# Autodesk Inventor assembly: Робот RRO 2021
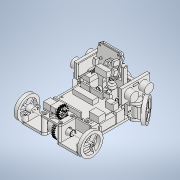
[picture p0: Inventor's stored thumbnail of the model, 180x180]
Saved by Autodesk Inventor 2020 (Build 240168000, 168)
## iProperties
Created: 2021-02-28
Part Number: Робот RRO 2021
Document SubType Name: Assembly
Designer: Антон
Author: Антон
## Documents named in this file (44)
- D:\Project\Robots\RRO 2021\Робот RRO 2021.iam
- D:\Project\Robots\RRO 2021\Body\Основа робота.ipt
- D:\Project\Robots\RRO 2021\Components\Кронштейн для двигателей серии N.ipt
- D:\Project\Robots\RRO 2021\Components\Servo SG90.ipt
- D:\Project\Robots\RRO 2021\Body\Основа рулевого механизма.ipt
- D:\Project\Robots\RRO 2021\Components\Подшипники\Подшипник 3 8 3.ipt
- D:\Project\Robots\RRO 2021\Components\Оси\Ось 3мм рулевого управления.ipt
- D:\Project\Robots\RRO 2021\Body\Деталь крепления диска к поворотному механизму.ipt
- D:\Project\Robots\RRO 2021\Components\Оси\Ось 3мм колеса.ipt
- D:\Project\Robots\RRO 2021\Body\Втулка между подшипниками рулевого управления.ipt
- D:\Project\Robots\RRO 2021\Components\Оси\Ось балки рулевого управления ведущая.ipt
- D:\Project\Robots\RRO 2021\Body\Балка рулевого управления ведущая.ipt
- D:\Project\Robots\RRO 2021\Body\Деталь крепления диска к поворотному механизму_ЗЕРКАЛО1.ipt
- D:\Project\Robots\RRO 2021\Body\Стойка под электроннику.ipt
- D:\Project\Robots\RRO 2021\Components\Arduino UNO.ipt
- D:\Project\Robots\RRO 2021\Body\Крепление камеры.ipt
- D:\Project\Robots\RRO 2021\Components\nVision lipo battery.ipt
- D:\Project\Robots\RRO 2021\Components\Micro Gearmotors.ipt
- D:\Project\Robots\RRO 2021\Components\Trackingcam (Applied robotics).ipt
- D:\Project\Robots\RRO 2021\Body\Стойка для камеры.ipt
- D:\Project\Robots\RRO 2021\Components\Подшипники\Подшипник 2 5 2,5.ipt
- D:\Project\Robots\RRO 2021\Components\Оси\Ось 2мм рулевой сервы.ipt
- D:\Project\Robots\RRO 2021\Body\Поворотный рычаг для сервы.ipt
- D:\Project\Robots\RRO 2021\Body\Крышка стойки подшипника 3мм.ipt
- D:\Project\Robots\RRO 2021\Body\Стойки камеры.ipt
- D:\Project\Robots\RRO 2021\Body\Съемная стойка сервы.ipt
- D:\Project\Robots\RRO 2021\Body\Крышка поворотного кулака.ipt
- D:\Project\Robots\RRO 2021\Components\Ultrasonic HC-SRO4.ipt
- D:\Project\Robots\RRO 2021\Body\Крышка аккумулятора.ipt
- D:\Project\Robots\RRO 2021\Body\Стойка подшипника 3мм.ipt
- D:\Project\Robots\RRO 2021\Components\Оси\Ось 3мм задняя.ipt
- D:\Project\Robots\RRO 2021\Body\Крепление ультрасоника.ipt
- D:\Project\Robots\RRO 2021\Body\Крепление ультрасоника вертикальная.ipt
- D:\Project\Robots\RRO 2021\Body\Крепление ультрасоника вертикальная_ЗЕРКАЛО.ipt
- D:\Project\Robots\RRO 2021\Components\Дифференциал.ipt
- D:\Project\Robots\RRO 2021\Body\Ведущая шестерня дифференециала.ipt
- D:\Project\Robots\RRO 2021\Components\Подшипники\Подшипник 10 15 4.ipt
- D:\Project\Robots\RRO 2021\Body\Переходник с дифференциала на ось 3мм.ipt
- D:\Project\Robots\RRO 2021\Components\Оси\Ось мотора серии N.ipt
- D:\Project\Robots\RRO 2021\Body\Крепление дифференциала.ipt
- D:\Project\Robots\RRO 2021\Body\Крепление двигателя2.ipt
- D:\Project\Robots\RRO 2021\Body\Проставка для двигателя.ipt
- D:\Project\Robots\RRO 2021\Components\Колесо D40 под ось моторов серии N.ipt
- D:\Project\Robots\RRO 2021\Body\Деталь основы рулевого управления.ipt
## Components (75 placed, 43 different names)
1. Основа робота:1 — Жесткий:138, Жесткий:152, Жесткий:153, Жесткий:189, Жесткий:190, Жесткий:195, Жесткий:203
2. Основа рулевого механизма:1 — Жесткий:45, С поворотом:161, Жесткий:181, Жесткий:186, Жесткий:195, Жесткий:201, Жесткий:202, Жесткий:204, Жесткий:208, Жесткий:209
3. Съемная стойка сервы:1 — Жесткий:186
4. Servo SG90:2 — Жесткий:181, С поворотом:163
5. Поворотный рычаг для сервы:1 — С поворотом:163, Жесткий:183
6. Подшипник 2*5*2.5:2 — С поворотом:162, Жесткий:183
7. Ось 2мм рулевой сервы:1 — С поворотом:24, С поворотом:162
8. Подшипник 2*5*2.5:1 — С поворотом:24, Жесткий:184
9. Балка рулевого управления:1 — С поворотом:35, С поворотом:36, Жесткий:184
10. Деталь основы рулевого управления:2 — Жесткий:208
11. Деталь основы рулевого управления:1 — Жесткий:209
12. Крышка аккумулятора:1 — Жесткий:108
13. nVision lipo battery:1 — Жесткий:54
14. Стойка под электроннику:1 — Жесткий:53, Жесткий:54, Жесткий:108, Жесткий:203
15. Arduino UNO:1 — Жесткий:53
16. Ось 3мм задняя:2 — Жесткий:165, Жесткий:197
17. Крепление двигателя2:1 — Жесткий:191, Жесткий:194
18. Переходник с дифференциала на ось 3мм:1 — Жесткий:165, Жесткий:171
19. Дифференциал:1 — С поворотом:158, Жесткий:166, ЗубчПер:1, Жесткий:171, С поворотом:164
20. Переходник с дифференциала на ось 3мм:2 — Жесткий:166, Жесткий:170
21. Ось 3мм задняя:1 — Жесткий:170, Жесткий:196
22. Колесо D40 под ось моторов серии N:1 — Жесткий:196
23. Колесо D40 под ось моторов серии N:2 — Жесткий:199
24. Колесо D40 под ось моторов серии N:4 — Жесткий:197
25. Колесо D40 под ось моторов серии N:3 — Жесткий:198
26. Стойка для камеры:1 — С поворотом:32, Жесткий:204
27. Крышка поворотного кулака:2 — Жесткий:137
28. Деталь крепления диска к поворотному механизму:1 — Жесткий:13, Жесткий:14, Жесткий:34, Жесткий:125, Жесткий:137
29. Втулка между подшипниками рулевого управления:1 — Жесткий:11, Жесткий:12
30. Крышка поворотного кулака:1 — Жесткий:136
31. Деталь крепления диска к поворотному механизму_ЗЕРКАЛО1:1 — Жесткий:37, Жесткий:38, Жесткий:39, Жесткий:44, Жесткий:136
32. Втулка между подшипниками рулевого управления:2
33. Кронштейн для двигателей серии N:1 — Жесткий:174, Жесткий:193
34. Micro Gearmotors:1 — С поворотом:160, Жесткий:174
35. Проставка для двигателя:1 — Жесткий:193, Жесткий:194
36. Ось мотора серии N:1 — С поворотом:160, Жесткий:192
37. Ведущая шестерня дифференециала:1 — ЗубчПер:1, Жесткий:192
38. Крышка стойки подшипника 3мм:1 — Жесткий:109, Жесткий:110
39. Подшипник 3*8*3:9 — Жесткий:109
40. Стойка подшипника 3мм:1 — Жесткий:110, Жесткий:153
41. Крепление дифференциала:1 — Жесткий:188, Жесткий:189, Жесткий:191
42. Подшипник 10 15 4:1 — С поворотом:158, Жесткий:188
43. Крепление дифференциала:2 — Жесткий:190
44. Подшипник 10 15 4:2 — С поворотом:164
45. Крышка стойки подшипника 3мм:4 — Жесткий:114, Жесткий:163
46. Подшипник 3*8*3:10 — Жесткий:163
47. Стойка подшипника 3мм:4 — Жесткий:114, Жесткий:152
48. Крепление ультрасоника вертикальная_ЗЕРКАЛО:1 — Жесткий:202, Жесткий:205
49. Ultrasonic HC-SRO4:3 — Жесткий:205
50. Ultrasonic HC-SRO4:1 — Жесткий:207
51. Крепление ультрасоника горизонтальное:1 — Жесткий:138, Жесткий:207
52. Крепление ультрасоника вертикальное:1 — Жесткий:201, Жесткий:206
53. Ultrasonic HC-SRO4:2 — Жесткий:206
54. Trackingcam (Applied robotics):1 — Жесткий:95, Жесткий:96, Жесткий:97, Жесткий:98
55. Стойки камеры:1 — Жесткий:98
56. Стойки камеры:2 — Жесткий:95, Жесткий:99
57. Стойки камеры:3 — Жесткий:97
58. Стойки камеры:4 — Жесткий:96
59. Крепление камеры:1 — С поворотом:32, Жесткий:99
60. Ось 3мм рулевого управления:3 — С поворотом:14, Жесткий:14
61. Ось 3мм колеса:1 — С поворотом:12, Жесткий:199
62. Ось 3мм рулевого управления:1 — С поворотом:13, Жесткий:13
63. Ось балки рулевого управления ведущая:2 — Жесткий:34, С поворотом:35
64. Подшипник 3*8*3:1 — Жесткий:12
65. Подшипник 3*8*3:2 — С поворотом:13, Жесткий:45
66. Подшипник 3*8*3:3 — С поворотом:14
67. Подшипник 3*8*3:4 — Жесткий:11, С поворотом:12, Жесткий:125
68. Ось 3мм колеса:2 — Жесткий:198
69. Ось 3мм рулевого управления:4 — С поворотом:16, Жесткий:44
70. Ось балки рулевого управления ведущая:1 — Жесткий:39, С поворотом:36
71. Ось 3мм рулевого управления:5 — Жесткий:37
72. Подшипник 3*8*3:7
73. Подшипник 3*8*3:8 — Жесткий:38
74. Подшипник 3*8*3:6 — С поворотом:16, С поворотом:161
75. Подшипник 3*8*3:5
## Relationships (77: WeldJoint 60, RevoluteJoint 16, RelateRotation 1)
- Жесткий:11 [WeldJoint]: Втулка между подшипниками рулевого управления:1 ↔ Подшипник 3*8*3:4
- Жесткий:12 [WeldJoint]: Втулка между подшипниками рулевого управления:1 ↔ Подшипник 3*8*3:1
- С поворотом:12 [RevoluteJoint]: Ось 3мм колеса:1 ↔ Подшипник 3*8*3:4
- С поворотом:13 [RevoluteJoint]: Ось 3мм рулевого управления:1 ↔ Подшипник 3*8*3:2
- С поворотом:14 [RevoluteJoint]: Ось 3мм рулевого управления:3 ↔ Подшипник 3*8*3:3
- Жесткий:13 [WeldJoint]: Деталь крепления диска к поворотному механизму:1 ↔ Ось 3мм рулевого управления:1
- Жесткий:14 [WeldJoint]: Деталь крепления диска к поворотному механизму:1 ↔ Ось 3мм рулевого управления:3
- [WeldJoint]: Втулка между подшипниками рулевого управления:2 ↔ Подшипник 3*8*3:8
- [WeldJoint]: Втулка между подшипниками рулевого управления:2 ↔ Подшипник 3*8*3:5
- [RevoluteJoint]: Ось 3мм колеса:2 ↔ Подшипник 3*8*3:8
- С поворотом:16 [RevoluteJoint]: Ось 3мм рулевого управления:4 ↔ Подшипник 3*8*3:6
- [RevoluteJoint]: Ось 3мм рулевого управления:5 ↔ Подшипник 3*8*3:7
- Жесткий:34 [WeldJoint]: Деталь крепления диска к поворотному механизму:1 ↔ Ось балки рулевого управления ведущая:2
- Жесткий:37 [WeldJoint]: Деталь крепления диска к поворотному механизму_ЗЕРКАЛО1:1 ↔ Ось 3мм рулевого управления:5
- Жесткий:38 [WeldJoint]: Деталь крепления диска к поворотному механизму_ЗЕРКАЛО1:1 ↔ Подшипник 3*8*3:8
- Жесткий:39 [WeldJoint]: Деталь крепления диска к поворотному механизму_ЗЕРКАЛО1:1 ↔ Ось балки рулевого управления ведущая:1
- Жесткий:44 [WeldJoint]: Деталь крепления диска к поворотному механизму_ЗЕРКАЛО1:1 ↔ Ось 3мм рулевого управления:4
- Жесткий:45 [WeldJoint]: Основа рулевого механизма:1 ↔ Подшипник 3*8*3:2
- Жесткий:53 [WeldJoint]: Стойка под электроннику:1 ↔ Arduino UNO:1
- Жесткий:54 [WeldJoint]: nVision lipo battery:1 ↔ Стойка под электроннику:1
- С поворотом:24 [RevoluteJoint]: Ось 2мм рулевой сервы:1 ↔ Подшипник 2*5*2.5:1
- С поворотом:32 [RevoluteJoint] (-0.15 mm): Стойка для камеры:1 ↔ Крепление камеры:1
- Жесткий:95 [WeldJoint]: Trackingcam (Applied robotics):1 ↔ Стойки камеры:2
- Жесткий:96 [WeldJoint]: Trackingcam (Applied robotics):1 ↔ Стойки камеры:4
- Жесткий:97 [WeldJoint]: Trackingcam (Applied robotics):1 ↔ Стойки камеры:3
- Жесткий:98 [WeldJoint]: Trackingcam (Applied robotics):1 ↔ Стойки камеры:1
- Жесткий:99 [WeldJoint]: Стойки камеры:2 ↔ Крепление камеры:1
- Жесткий:108 [WeldJoint]: Крышка аккумулятора:1 ↔ Стойка под электроннику:1
- Жесткий:109 [WeldJoint] (-0.05 mm): Крышка стойки подшипника 3мм:1 ↔ Подшипник 3*8*3:9
- Жесткий:110 [WeldJoint]: Крышка стойки подшипника 3мм:1 ↔ Стойка подшипника 3мм:1
- Жесткий:114 [WeldJoint]: Крышка стойки подшипника 3мм:4 ↔ Стойка подшипника 3мм:4
- Жесткий:125 [WeldJoint]: Деталь крепления диска к поворотному механизму:1 ↔ Подшипник 3*8*3:4
- С поворотом:35 [RevoluteJoint]: Балка рулевого управления:1 ↔ Ось балки рулевого управления ведущая:2
- С поворотом:36 [RevoluteJoint]: Балка рулевого управления:1 ↔ Ось балки рулевого управления ведущая:1
- Жесткий:136 [WeldJoint]: Крышка поворотного кулака:1 ↔ Деталь крепления диска к поворотному механизму_ЗЕРКАЛО1:1
- Жесткий:137 [WeldJoint]: Крышка поворотного кулака:2 ↔ Деталь крепления диска к поворотному механизму:1
- Жесткий:138 [WeldJoint]: Основа робота:1 ↔ Крепление ультрасоника горизонтальное:1
- Жесткий:152 [WeldJoint]: Основа робота:1 ↔ Стойка подшипника 3мм:4
- Жесткий:153 [WeldJoint]: Основа робота:1 ↔ Стойка подшипника 3мм:1
- С поворотом:158 [RevoluteJoint] (-1 mm): Дифференциал:1 ↔ Подшипник 10 15 4:1
- Жесткий:163 [WeldJoint] (-0.05 mm): Крышка стойки подшипника 3мм:4 ↔ Подшипник 3*8*3:10
- Жесткий:165 [WeldJoint]: Ось 3мм задняя:2 ↔ Переходник с дифференциала на ось 3мм:1
- Жесткий:166 [WeldJoint]: Дифференциал:1 ↔ Переходник с дифференциала на ось 3мм:2
- Жесткий:170 [WeldJoint]: Переходник с дифференциала на ось 3мм:2 ↔ Ось 3мм задняя:1
- ЗубчПер:1 [RelateRotation] (2 ul): Дифференциал:1 ↔ Ведущая шестерня дифференециала:1
- С поворотом:160 [RevoluteJoint]: Micro Gearmotors:1 ↔ Ось мотора серии N:1
- Жесткий:171 [WeldJoint]: Переходник с дифференциала на ось 3мм:1 ↔ Дифференциал:1
- Жесткий:174 [WeldJoint]: Кронштейн для двигателей серии N:1 ↔ Micro Gearmotors:1
- С поворотом:161 [RevoluteJoint]: Основа рулевого механизма:1 ↔ Подшипник 3*8*3:6
- Жесткий:181 [WeldJoint]: Основа рулевого механизма:1 ↔ Servo SG90:2
- С поворотом:162 [RevoluteJoint]: Подшипник 2*5*2.5:2 ↔ Ось 2мм рулевой сервы:1
- С поворотом:163 [RevoluteJoint]: Servo SG90:2 ↔ Поворотный рычаг для сервы:1
- Жесткий:183 [WeldJoint]: Поворотный рычаг для сервы:1 ↔ Подшипник 2*5*2.5:2
- Жесткий:184 [WeldJoint]: Подшипник 2*5*2.5:1 ↔ Балка рулевого управления:1
- Жесткий:186 [WeldJoint]: Основа рулевого механизма:1 ↔ Съемная стойка сервы:1
- Жесткий:188 [WeldJoint]: Крепление дифференциала:1 ↔ Подшипник 10 15 4:1
- С поворотом:164 [RevoluteJoint] (-1 mm): Дифференциал:1 ↔ Подшипник 10 15 4:2
- Жесткий:189 [WeldJoint]: Основа робота:1 ↔ Крепление дифференциала:1
- Жесткий:190 [WeldJoint]: Основа робота:1 ↔ Крепление дифференциала:2
- Жесткий:191 [WeldJoint]: Крепление двигателя2:1 ↔ Крепление дифференциала:1
- Жесткий:192 [WeldJoint]: Ось мотора серии N:1 ↔ Ведущая шестерня дифференециала:1
- Жесткий:193 [WeldJoint]: Кронштейн для двигателей серии N:1 ↔ Проставка для двигателя:1
- Жесткий:194 [WeldJoint]: Крепление двигателя2:1 ↔ Проставка для двигателя:1
- Жесткий:195 [WeldJoint]: Основа робота:1 ↔ Основа рулевого механизма:1
- Жесткий:196 [WeldJoint]: Ось 3мм задняя:1 ↔ Колесо D40 под ось моторов серии N:1
- Жесткий:197 [WeldJoint]: Ось 3мм задняя:2 ↔ Колесо D40 под ось моторов серии N:4
- Жесткий:198 [WeldJoint]: Колесо D40 под ось моторов серии N:3 ↔ Ось 3мм колеса:2
- Жесткий:199 [WeldJoint]: Колесо D40 под ось моторов серии N:2 ↔ Ось 3мм колеса:1
- Жесткий:201 [WeldJoint]: Основа рулевого механизма:1 ↔ Крепление ультрасоника вертикальное:1
- Жесткий:202 [WeldJoint]: Основа рулевого механизма:1 ↔ Крепление ультрасоника вертикальная_ЗЕРКАЛО:1
- Жесткий:203 [WeldJoint]: Основа робота:1 ↔ Стойка под электроннику:1
- Жесткий:204 [WeldJoint] (-0.1 mm): Основа рулевого механизма:1 ↔ Стойка для камеры:1
- Жесткий:205 [WeldJoint]: Крепление ультрасоника вертикальная_ЗЕРКАЛО:1 ↔ Ultrasonic HC-SRO4:3
- Жесткий:206 [WeldJoint]: Крепление ультрасоника вертикальное:1 ↔ Ultrasonic HC-SRO4:2
- Жесткий:207 [WeldJoint]: Ultrasonic HC-SRO4:1 ↔ Крепление ультрасоника горизонтальное:1
- Жесткий:208 [WeldJoint]: Основа рулевого механизма:1 ↔ Деталь основы рулевого управления:2
- Жесткий:209 [WeldJoint]: Основа рулевого механизма:1 ↔ Деталь основы рулевого управления:1
## Named parameters: d71_d54 = 0 mm, d72_d55 = -34.721681 deg, d73_d56 = 0 mm, d74_d57 = -172.249559 deg, d75_d60 = 180 deg, d76_d61 = 0 deg, d79_d47 = 0 mm, d80_d48 = 0 mm, d81_d49 = 0 mm, d82_d50 = 0 deg
